# Autodesk Inventor assembly: outer
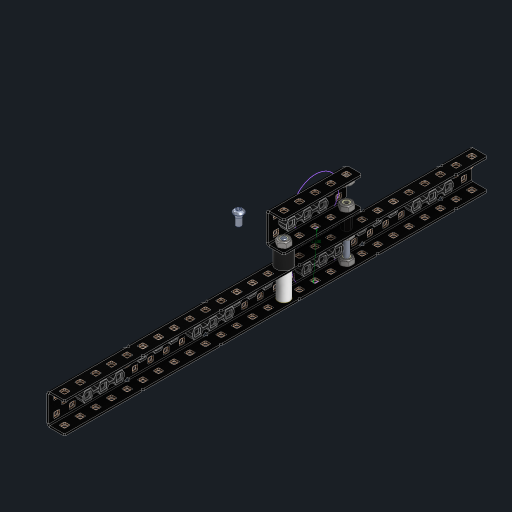
[picture p0: Inventor's stored thumbnail of the model, 512x512]
Saved by Autodesk Inventor 2024 (Build 280153000, 153)
## iProperties
Created: 2024-03-11
Part Number: outer
Document SubType Name: Assembly
Designer: Averey Ku
Author: Averey Ku
## Documents named in this file (15)
- D:\vex_robotics\hardware\cad\eca\chassis\drivebay\outer.iam
- D:\vex_robotics\hardware\cad\VEX-CAD-Inventor-1.41\Structure\C Channel\Aluminum 1x2x1\Alu C 1x2x1x27.ipt
- D:\vex_robotics\hardware\cad\VEX-CAD-Inventor-1.41\Motion\Shaft LS\Bearing Flat Low Profile.ipt
- D:\vex_robotics\hardware\cad\VEX-CAD-Inventor-1.41\Motion\Spacers\Spacer Nylon .500 OD\NSpacer Black .500 OD x .500.ipt
- D:\vex_robotics\hardware\cad\VEX-CAD-Inventor-1.41\Motion\Spacers\Spacer Nylon .500 OD.ipt
- D:\vex_robotics\hardware\cad\VEX-CAD-Inventor-1.41\Structure\C Channel\Aluminum 1x2x1\Alu C 1x2x1x5.ipt
- D:\vex_robotics\hardware\cad\VEX-CAD-Inventor-1.41\Structure\Hardware\Screw Steel - Star\SScrew Star Smooth 1.750.ipt
- D:\vex_robotics\hardware\cad\VEX-CAD-Inventor-1.41\Structure\Hardware\Screw Steel - Star.ipt
- D:\vex_robotics\hardware\cad\VEX-CAD-Inventor-1.41\Structure\Hardware\Nut Thin Nylock.ipt
- D:\vex_robotics\hardware\cad\hardware\.375 OD Aluminum Spacer 0.875.ipt
- D:\vex_robotics\hardware\cad\VEX-CAD-Inventor-1.41\Structure\Hardware\Screw Steel - Star\SScrew Star Smooth 1.250.ipt
- D:\vex_robotics\hardware\cad\VEX-CAD-Inventor-1.41\Structure\Standoff\Standoff .50.ipt
- D:\vex_robotics\hardware\cad\VEX-CAD-Inventor-1.41\Structure\Standoff.ipt
- D:\vex_robotics\hardware\cad\VEX-CAD-Inventor-1.41\Structure\Hardware\Screw Shoulder Robosource\SScrew Shoulder Smooth .375 x .12.ipt
- D:\vex_robotics\hardware\cad\VEX-CAD-Inventor-1.41\Structure\Hardware\Screw Shoulder Robosource.ipt
## Components (21 placed, 10 different names)
1. Alu C 1x2x1x27:1 — Insert:1, Mate:1, Insert:2, Mate:2, Insert:3, Mate:3, Insert:5, Mate:5, Insert:6, Mate:6, Insert:7, Mate:7, Insert:10, Mate:10, Insert:12, Mate:12, Insert:13, Insert:14, Insert:16, Insert:17, Insert:18, Insert:19, Insert:20
2. Bearing Flat Low Profile:1 — Insert:1, Mate:1
3. Bearing Flat Low Profile:2 — Insert:2, Mate:2
4. Bearing Flat Low Profile:3 — Insert:3, Mate:3
5. Bearing Flat Low Profile:4 — Insert:10, Mate:10
6. Bearing Flat Low Profile:5 — Insert:5, Mate:5
7. Bearing Flat Low Profile:6 — Insert:6, Mate:6
8. Bearing Flat Low Profile:7 — Insert:7, Mate:7
9. Bearing Flat Low Profile:8 — Insert:11, Mate:11
10. NSpacer Black .500 OD x .500:2 — Insert:14
11. Alu C 1x2x1x5:1 — Insert:11, Mate:11, Insert:12, Mate:12, Insert:15, Insert:21, Insert:22
12. SScrew Star Smooth 1.750:1 — Insert:13
13. Nut Thin Nylock:1 — Insert:15
14. .375 OD Aluminum Spacer 0.875:1 — Insert:16
15. SScrew Star Smooth 1.250:2 — Insert:17
16. Nut Thin Nylock:2 — Insert:19
17. Nut Thin Nylock:3 — Insert:18
18. Standoff .50:1 — Insert:20
19. Nut Thin Nylock:4 — Insert:22
20. Nut Thin Nylock:5 — Insert:21
21. SScrew Shoulder Smooth .375 x .12:1
## Relationships (28: Insert 19, Mate 9)
- Insert:1: Alu C 1x2x1x27:1 ↔ Bearing Flat Low Profile:1
- Mate:1: Alu C 1x2x1x27:1 ↔ Bearing Flat Low Profile:1
- Insert:2: Alu C 1x2x1x27:1 ↔ Bearing Flat Low Profile:2
- Mate:2: Alu C 1x2x1x27:1 ↔ Bearing Flat Low Profile:2
- Insert:3: Alu C 1x2x1x27:1 ↔ Bearing Flat Low Profile:3
- Mate:3: Alu C 1x2x1x27:1 ↔ Bearing Flat Low Profile:3
- Insert:5: Alu C 1x2x1x27:1 ↔ Bearing Flat Low Profile:5
- Mate:5: Alu C 1x2x1x27:1 ↔ Bearing Flat Low Profile:5
- Insert:6: Alu C 1x2x1x27:1 ↔ Bearing Flat Low Profile:6
- Mate:6: Alu C 1x2x1x27:1 ↔ Bearing Flat Low Profile:6
- Insert:7: Alu C 1x2x1x27:1 ↔ Bearing Flat Low Profile:7
- Mate:7: Alu C 1x2x1x27:1 ↔ Bearing Flat Low Profile:7
- Insert:10: Alu C 1x2x1x27:1 ↔ Bearing Flat Low Profile:4
- Mate:10: Alu C 1x2x1x27:1 ↔ Bearing Flat Low Profile:4
- Insert:11: Bearing Flat Low Profile:8 ↔ Alu C 1x2x1x5:1
- Mate:11: Bearing Flat Low Profile:8 ↔ Alu C 1x2x1x5:1
- Insert:12 (12.7 mm): Alu C 1x2x1x27:1 ↔ Alu C 1x2x1x5:1
- Mate:12: Alu C 1x2x1x27:1 ↔ Alu C 1x2x1x5:1
- Insert:13: Alu C 1x2x1x27:1 ↔ SScrew Star Smooth 1.750:1
- Insert:14: Alu C 1x2x1x27:1 ↔ NSpacer Black .500 OD x .500:2
- Insert:15: Alu C 1x2x1x5:1 ↔ Nut Thin Nylock:1
- Insert:16: Alu C 1x2x1x27:1 ↔ .375 OD Aluminum Spacer 0.875:1
- Insert:17: Alu C 1x2x1x27:1 ↔ SScrew Star Smooth 1.250:2
- Insert:18: Alu C 1x2x1x27:1 ↔ Nut Thin Nylock:3
- Insert:19: Alu C 1x2x1x27:1 ↔ Nut Thin Nylock:2
- Insert:20: Alu C 1x2x1x27:1 ↔ Standoff .50:1
- Insert:21: Alu C 1x2x1x5:1 ↔ Nut Thin Nylock:5
- Insert:22: Alu C 1x2x1x5:1 ↔ Nut Thin Nylock:4
